# Autodesk Inventor assembly: Slide_Plate_RFinish
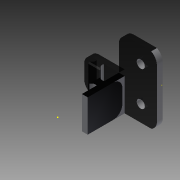
[picture p0: Inventor's stored thumbnail of the model, 180x180]
Saved by Autodesk Inventor 2014 (Build 180170000, 170)
## iProperties
Created: 2015-01-31
Part Number: Slide_Plate_RFinish
Document SubType Name: Assembly
Designer: Owner
Author: Owner
## Documents named in this file (3)
- C:\Users\Owner\Desktop\Lockdown Programs\Slide_Plate_RFinish.iam
- C:\Users\Owner\Desktop\Lockdown Programs\Slide_Plate_RExtResize.ipt
- C:\Users\Owner\Desktop\Lockdown Programs\Slide_Plate_RTslot.ipt
## Components (2 placed, 2 different names)
1. Slide_Plate_RExtResize:1 — Rigid:1, Rigid:2
2. Slide_Plate_RTslot:1 — Rigid:1, Rigid:2
## Relationships (2: WeldJoint 2)
- Rigid:1 [WeldJoint]: Slide_Plate_RExtResize:1 ↔ Slide_Plate_RTslot:1
- Rigid:2 [WeldJoint]: Slide_Plate_RExtResize:1 ↔ Slide_Plate_RTslot:1
